# Autodesk Inventor assembly: cage nut m6
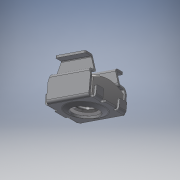
[picture p0: Inventor's stored thumbnail of the model, 180x180]
Saved by Autodesk Inventor 2016 (Build 200138000, 138)
## iProperties
Created: 2015-10-24
Part Number: cage nut m6
Document SubType Name: Assembly
Designer: jeremyhale
Author: jeremyhale
## Documents named in this file (3)
- \\psf\Home\Documents\Poorhouse\git\p0001\cage nut m6.iam
- \\psf\Home\Documents\Poorhouse\git\p0001\cage nut m6.ipt
- \\psf\Home\Documents\Inventor\Content Center Files\R2016\en-US\DIN 557\DIN 557 - M6 x 10.ipt
## Components (2 placed, 2 different names)
1. cage nut m6:1 — Insert:1, Angle:1
2. DIN 557 M6:1 — Insert:1, Angle:1
## Relationships (2: Insert 1, Angle 1)
- Insert:1: cage nut m6:1 ↔ DIN 557 M6:1
- Angle:1 (0 deg): cage nut m6:1 ↔ DIN 557 M6:1
